# Autodesk Inventor assembly: stepover_2
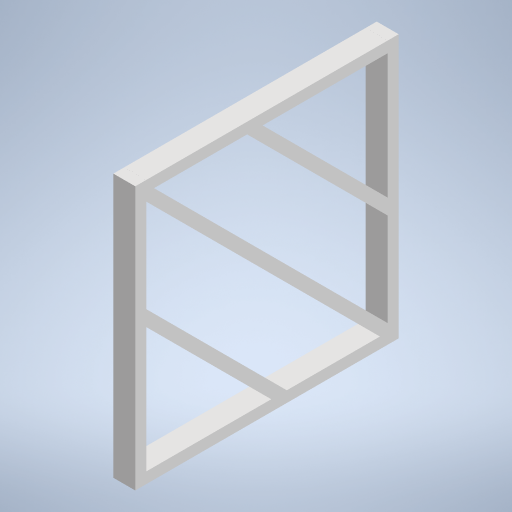
[picture p0: Inventor's stored thumbnail of the model, 512x512]
Saved by Autodesk Inventor 2024.2 (Build 282272000, 272)
## iProperties
Created: 2024-01-16
Part Number: stepover_2
Document SubType Name: Assembly
Designer: HukoOo
Author: HukoOo
## Documents named in this file (5)
- E:\OneDrive - 성균관대학교\Projects\2024 ICRA QRC 대회\모델\stepover_2.iam
- E:\OneDrive - 성균관대학교\Projects\2024 ICRA QRC 대회\모델\board_50x100x1100.ipt
- E:\OneDrive - 성균관대학교\Projects\2024 ICRA QRC 대회\모델\board_50x100x1200.ipt
- E:\OneDrive - 성균관대학교\Projects\2024 ICRA QRC 대회\모델\stepover_part1.ipt
- E:\OneDrive - 성균관대학교\Projects\2024 ICRA QRC 대회\모델\stepover_part2.ipt
## Components (6 placed, 4 different names)
1. board_50x100x1100:1 — 메이트:2, 플러쉬:3, 플러쉬:6, 플러쉬:8
2. board_50x100x1100:2 — 메이트:3, 플러쉬:4, 플러쉬:5, 플러쉬:7
3. board_50x100x1200:1 — 플러쉬:1, 플러쉬:2, 메이트:1, 메이트:2, 플러쉬:3, 메이트:3, 플러쉬:4, 플러쉬:5, 플러쉬:6
4. board_50x100x1200:2 — 플러쉬:1, 플러쉬:2, 메이트:1
5. stepover_part1:1 — 플러쉬:7
6. stepover_part2:1 — 플러쉬:8
## Relationships (11: Flush 8, Mate 3)
- 플러쉬:1 [Flush]: board_50x100x1200:1 ↔ board_50x100x1200:2
- 플러쉬:2 [Flush]: board_50x100x1200:1 ↔ board_50x100x1200:2
- 메이트:1 [Mate] (1100 mm): board_50x100x1200:1 ↔ board_50x100x1200:2
- 메이트:2 [Mate]: board_50x100x1100:1 ↔ board_50x100x1200:1
- 플러쉬:3 [Flush]: board_50x100x1100:1 ↔ board_50x100x1200:1
- 메이트:3 [Mate]: board_50x100x1100:2 ↔ board_50x100x1200:1
- 플러쉬:4 [Flush]: board_50x100x1100:2 ↔ board_50x100x1200:1
- 플러쉬:5 [Flush]: board_50x100x1100:2 ↔ board_50x100x1200:1
- 플러쉬:6 [Flush]: board_50x100x1100:1 ↔ board_50x100x1200:1
- 플러쉬:7 [Flush]: board_50x100x1100:2 ↔ stepover_part1:1
- 플러쉬:8 [Flush]: board_50x100x1100:1 ↔ stepover_part2:1
